# Autodesk Inventor assembly: NewClaw
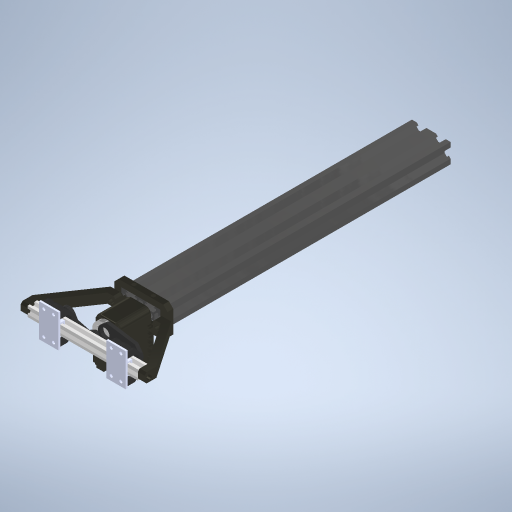
[picture p0: Inventor's stored thumbnail of the model, 512x512]
Saved by Autodesk Inventor 2024.3 (Build 283343000, 343)
## iProperties
Created: 2025-01-07
Part Number: NewClaw
Document SubType Name: Assembly
Designer: migue
Author: migue
## Documents named in this file (12)
- C:\Users\migue\Documents\GitHub\RobotCartesiano\DiseñoMecánico\Assemblies\NewClaw.iam
- C:\Users\migue\Documents\GitHub\RobotCartesiano\DiseñoMecánico\AcrylicPieces\ServoCarrier.ipt
- C:\Users\migue\Documents\GitHub\RobotCartesiano\DiseñoMecánico\Axis\AxisZ\MovingPlate\AP-ZClaw.ipt
- C:\Users\migue\Documents\GitHub\RobotCartesiano\DiseñoMecánico\Axis\AxisZ\MovingPlate\AP10x10.ipt
- C:\Users\migue\Documents\GitHub\RobotCartesiano\DiseñoMecánico\Axis\AxisZ\MovingPlate\MechanismArm.ipt
- C:\Users\migue\Documents\GitHub\RobotCartesiano\DiseñoMecánico\Motors\DynamixelAX12A\Pieces\AX12 middle.STEP.ipt
- C:\Users\migue\Documents\GitHub\RobotCartesiano\DiseñoMecánico\Motors\DynamixelAX12A\Pieces\AX12 Back.STEP.ipt
- C:\Users\migue\Documents\GitHub\RobotCartesiano\DiseñoMecánico\Motors\DynamixelAX12A\Pieces\AX12 Front.STEP.ipt
- C:\Users\migue\Documents\GitHub\RobotCartesiano\DiseñoMecánico\Motors\DynamixelAX12A\Pieces\Axel.STEP.ipt
- C:\Users\migue\Documents\GitHub\RobotCartesiano\DiseñoMecánico\Axis\AxisZ\MovingPlate\GripperSupport.ipt
- C:\Users\migue\Documents\GitHub\RobotCartesiano\DiseñoMecánico\Axis\AxisZ\MovingPlate\SliderPiece.ipt
- C:\Users\migue\Documents\GitHub\RobotCartesiano\DiseñoMecánico\Axis\AxisZ\MovingPlate\HoldingArms.ipt
## Components (15 placed, 11 different names)
1. ServoCarrier:1 — Mate:1, Flush:1, Mate:2, Mate:24
2. AP-ZClaw:1 — Mate:1, Flush:1, Mate:2, Flush:6, Flush:7, Flush:12
3. MechanismArm:1 — Mate:7, Mate:8, Mate:23
4. MechanismArm:2 — Mate:9, Mate:10, Mate:21, Mate:22
5. Axel.STEP:1 — Mate:5, Mate:6, Mate:7, Mate:8, Mate:9, Mate:10
6. GripperSupport:4 — Mate:11, Mate:12, Mate:13, Mate:23
7. GripperSupport:5 — Mate:14, Mate:15, Mate:16, Mate:21, Mate:22
8. SliderPiece:1 — Mate:11, Mate:12, Mate:13, Mate:25, Mate:26
9. SliderPiece:2 — Mate:14, Mate:15, Mate:16, Mate:27, Mate:28
10. AP10x10:1 — Flush:6, Mate:25, Mate:26, Mate:27, Mate:28, Flush:7, Mate:29, Flush:8, Flush:9, Mate:30, Flush:10, Flush:11
11. HoldingArms:1 — Mate:29, Flush:8, Flush:9
12. HoldingArms:2 — Mate:30, Flush:10, Flush:11
13. AX12 middle.STEP:1 — Mate:3, Flush:2, Flush:3, Flush:4, Mate:4, Flush:5, Flush:12
14. AX12 Back.STEP:1 — Mate:3, Flush:2, Flush:3, Mate:24
15. AX12 Front.STEP:1 — Flush:4, Mate:4, Flush:5, Mate:5, Mate:6
## Relationships (38: Mate 26, Flush 12)
- Mate:1: ServoCarrier:1 ↔ AP-ZClaw:1
- Flush:1: ServoCarrier:1 ↔ AP-ZClaw:1
- Mate:2: ServoCarrier:1 ↔ AP-ZClaw:1
- Mate:3: AX12 middle.STEP:1 ↔ AX12 Back.STEP:1
- Flush:2: AX12 middle.STEP:1 ↔ AX12 Back.STEP:1
- Flush:3: AX12 middle.STEP:1 ↔ AX12 Back.STEP:1
- Flush:4: AX12 middle.STEP:1 ↔ AX12 Front.STEP:1
- Mate:4: AX12 middle.STEP:1 ↔ AX12 Front.STEP:1
- Flush:5: AX12 middle.STEP:1 ↔ AX12 Front.STEP:1
- Mate:5: Axel.STEP:1 ↔ AX12 Front.STEP:1
- Mate:6: Axel.STEP:1 ↔ AX12 Front.STEP:1
- Mate:7: MechanismArm:1 ↔ Axel.STEP:1
- Mate:8: MechanismArm:1 ↔ Axel.STEP:1
- Mate:9: MechanismArm:2 ↔ Axel.STEP:1
- Mate:10: MechanismArm:2 ↔ Axel.STEP:1
- Mate:11: GripperSupport:4 ↔ SliderPiece:1
- Mate:12: GripperSupport:4 ↔ SliderPiece:1
- Mate:13: GripperSupport:4 ↔ SliderPiece:1
- Mate:14: GripperSupport:5 ↔ SliderPiece:2
- Mate:15: GripperSupport:5 ↔ SliderPiece:2
- Mate:16: GripperSupport:5 ↔ SliderPiece:2
- Mate:21: MechanismArm:2 ↔ GripperSupport:5
- Mate:22: MechanismArm:2 ↔ GripperSupport:5
- Mate:23: MechanismArm:1 ↔ GripperSupport:4
- Mate:24: ServoCarrier:1 ↔ AX12 Back.STEP:1
- Flush:6 (-5 mm): AP-ZClaw:1 ↔ AP10x10:1
- Mate:25: SliderPiece:1 ↔ AP10x10:1
- Mate:26: SliderPiece:1 ↔ AP10x10:1
- Mate:27: SliderPiece:2 ↔ AP10x10:1
- Mate:28: SliderPiece:2 ↔ AP10x10:1
- Flush:7 (-37 mm): AP-ZClaw:1 ↔ AP10x10:1
- Mate:29: AP10x10:1 ↔ HoldingArms:1
- Flush:8: AP10x10:1 ↔ HoldingArms:1
- Flush:9: AP10x10:1 ↔ HoldingArms:1
- Mate:30: AP10x10:1 ↔ HoldingArms:2
- Flush:10: AP10x10:1 ↔ HoldingArms:2
- Flush:11: AP10x10:1 ↔ HoldingArms:2
- Flush:12: AP-ZClaw:1 ↔ AX12 middle.STEP:1
